# Autodesk Inventor assembly: 0701 ASY GBK wall shield Center 4
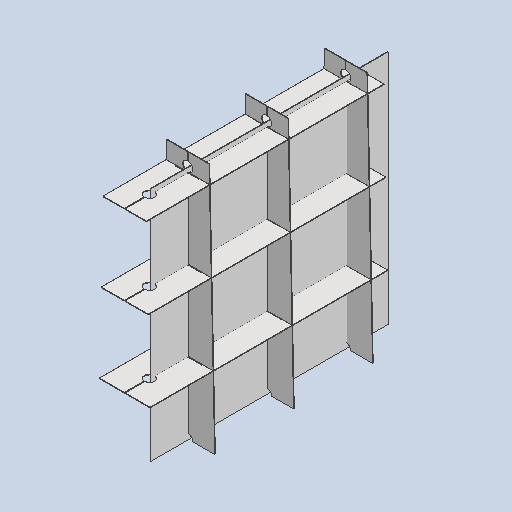
[picture p0: Inventor's stored thumbnail of the model, 512x512]
Saved by Autodesk Inventor 2026.2 (Build 302298000, 298)
## iProperties
Created: 2026-05-19
Part Number: 0701 ASY GBK wall shield Center 4
Document SubType Name: Assembly
Designer: pokla
Mass: 152628 g
Surface Area: 99280.6 cm^2
Volume: 19443.1 cm^3
Density: 7.85 g/cm^3
Author: admin
## Documents named in this file (6)
- C:\Users\admin\Documents\Inventor\GBK-Gubkinskiy\0701 ASY GBK wall shield Center 4.iam
- C:\Users\admin\Documents\Inventor\GBK-Gubkinskiy\0711 GBK Center rib 2.ipt
- C:\Users\admin\Documents\Inventor\GBK-Gubkinskiy\0713 GBK stringer C1.ipt
- C:\Users\admin\Documents\Inventor\GBK-Gubkinskiy\0714 GBK stringer C2.ipt
- C:\Users\admin\Documents\Inventor\GBK-Gubkinskiy\0715 GBK stringer C3.ipt
- C:\Users\admin\Documents\Inventor\GBK-Gubkinskiy\010.7 GBK shield.ipt
## Components (13 placed, 5 different names)
1. 0713 GBK stringer C1:1 — Rigid:1
2. 0714 GBK stringer C2:1 — Rigid:2
3. 0715 GBK stringer C3:1 — Rigid:3
4. 0713 GBK stringer C1:2 — Rigid:6
5. 0714 GBK stringer C2:2 — Rigid:5
6. 0715 GBK stringer C3:2 — Rigid:4
7. 010.7 GBK shield:1 — Mate:7, Mate:8
8. 0711 GBK Center rib 2:1 — Flush:4, Rigid:1, Rigid:2, Rigid:3, Mate:6
9. 0711 GBK Center rib 2:2 — Flush:4, Mate:5, Rigid:4, Rigid:5, Rigid:6
10. 0711 GBK Center rib 2:3
11. 0711 GBK Center rib 2:4
12. 0711 GBK Center rib 2:5
13. 0711 GBK Center rib 2:6
## Component patterns: (3 elements, first: 0711 GBK Center rib 2:1 + 0711 GBK Center rib 2:2)
## Relationships (11: WeldJoint 6, Mate 4, Flush 1)
- Flush:4: 0711 GBK Center rib 2:1 ↔ 0711 GBK Center rib 2:2
- Rigid:1 [WeldJoint] (4 mm): 0713 GBK stringer C1:1 ↔ 0711 GBK Center rib 2:1
- Rigid:2 [WeldJoint] (4 mm): 0714 GBK stringer C2:1 ↔ 0711 GBK Center rib 2:1
- Rigid:3 [WeldJoint] (4 mm): 0715 GBK stringer C3:1 ↔ 0711 GBK Center rib 2:1
- Mate:5: 0711 GBK Center rib 2:2
- Mate:6: 0711 GBK Center rib 2:1
- Rigid:4 [WeldJoint] (4 mm): 0715 GBK stringer C3:2 ↔ 0711 GBK Center rib 2:2
- Rigid:5 [WeldJoint] (4 mm): 0714 GBK stringer C2:2 ↔ 0711 GBK Center rib 2:2
- Rigid:6 [WeldJoint] (4 mm): 0713 GBK stringer C1:2 ↔ 0711 GBK Center rib 2:2
- Mate:7: 010.7 GBK shield:1
- Mate:8: 010.7 GBK shield:1
